# Autodesk Inventor assembly: dual_motor_turret
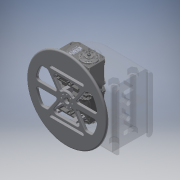
[picture p0: Inventor's stored thumbnail of the model, 180x180]
Saved by Autodesk Inventor 2018 (Build 220112000, 112)
## iProperties
Created: 2018-04-26
Part Number: dual_motor_turret
Document SubType Name: Assembly
Designer: mshaw2
Author: mshaw2
## Documents named in this file (5)
- C:\Users\mshaw2\OneDrive - University of Plymouth\ROCO224\dual_motor_turret.iam
- C:\Users\mshaw2\OneDrive - University of Plymouth\ROCO224\ENS_SERVO-RX-28.iam
- C:\Users\mshaw2\OneDrive - University of Plymouth\ROCO224\arm_segment_1_1a2.ipt
- C:\Users\mshaw2\OneDrive - University of Plymouth\ROCO224\arm_segment_1_1b2.ipt
- C:\Users\mshaw2\OneDrive - University of Plymouth\ROCO224\base_turret_v3.ipt
## Components (5 placed, 4 different names)
1. ENS_SERVO-RX-28:1 [sub-assembly] — Rigid:1, Rotational:1, Rigid:4
2. ENS_SERVO-RX-28:2 [sub-assembly] — Rigid:1
3. arm_segment_1_1a2:1 — Rotational:1, Rigid:3
4. arm_segment_1_1b2:1 — Rigid:3
5. base_turret_v3:1 — Rigid:4
## Relationships (4: WeldJoint 3, RevoluteJoint 1)
- Rigid:1 [WeldJoint] (0.5 mm): ENS_SERVO-RX-28:1 ↔ ENS_SERVO-RX-28:2
- Rotational:1 [RevoluteJoint] (0.25 mm): ENS_SERVO-RX-28:1 ↔ arm_segment_1_1a2:1
- Rigid:3 [WeldJoint]: arm_segment_1_1a2:1 ↔ arm_segment_1_1b2:1
- Rigid:4 [WeldJoint]: ENS_SERVO-RX-28:1 ↔ base_turret_v3:1
